# Autodesk Inventor assembly: HorquillaSuperior
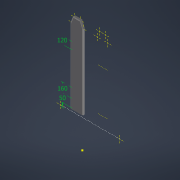
[picture p0: Inventor's stored thumbnail of the model, 180x180]
Saved by Autodesk Inventor 2022 (Build 260153000, 153)
## iProperties
Created: 2021-09-29
Part Number: HorquillaSuperior
Material: Generic
Document SubType Name: Assembly
Designer: Andres
Mass: 15301.1 g
Surface Area: 8967.62 cm^2
Volume: 1949.18 cm^3
Density: 7.85 g/cm^3
_SolveAssemblyDoc: Frame Generator Solve Assembly
_Version: 25.0.0
Author: Andres
## Documents named in this file (4)
- D:\Documentos\15.PUCP_2021-2\[PDM] Proyecto de Diseño Mecatrónico\ProyectoGIT\ProyectoRobotPallet\HorquillaSuperior\HorquillaSuperior.iam
- D:\Documentos\15.PUCP_2021-2\[PDM] Proyecto de Diseño Mecatrónico\ProyectoGIT\ProyectoRobotPallet\HorquillaSuperior\HorquillaSuperior.ipt
- D:\Documentos\15.PUCP_2021-2\[PDM] Proyecto de Diseño Mecatrónico\ProyectoGIT\ProyectoRobotPallet\HorquillaSuperior\HorquillaSuperior\Frame\Frame_HorqSup.iam
- D:\Documentos\15.PUCP_2021-2\[PDM] Proyecto de Diseño Mecatrónico\ProyectoGIT\ProyectoRobotPallet\HorquillaSuperior\PlanchaHorqSup.ipt
## Components (3 placed, 3 different names)
1. HorquillaSuperior:1
2. Frame_HorqSup:1 [sub-assembly] — Flush:1
3. PlanchaHorqSup:1 — Flush:1
## Relationships (1: Flush 1)
- Flush:1: Frame_HorqSup:1 ↔ PlanchaHorqSup:1
